# Autodesk Inventor assembly: Whales_Project
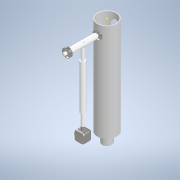
[picture p0: Inventor's stored thumbnail of the model, 180x180]
Saved by Autodesk Inventor 2020 (Build 240168000, 168)
## iProperties
Created: 2021-11-29
Part Number: Whales_Project
Document SubType Name: Assembly
Designer: Emrah BAYRAM
Author: Emrah BAYRAM
## Documents named in this file (11)
- C:\Users\umuro\OneDrive - ikc.edu.tr\Home - Library_Umur\E\Education\2020-2024_Mechatronics\Lessons\MEE203-DINAMIK\Whales_Dynamics_Project\Drawings\Assembly2.iam
- C:\Users\umuro\OneDrive - ikc.edu.tr\Home - Library_Umur\E\Education\2020-2024_Mechatronics\Lessons\MEE203-DINAMIK\Whales_Dynamics_Project\Drawings\Platform.ipt
- C:\Users\umuro\OneDrive - ikc.edu.tr\Home - Library_Umur\E\Education\2020-2024_Mechatronics\Lessons\MEE203-DINAMIK\Whales_Dynamics_Project\Drawings\Hammer.ipt
- C:\Users\umuro\OneDrive - ikc.edu.tr\Home - Library_Umur\E\Education\2020-2024_Mechatronics\Lessons\MEE203-DINAMIK\Whales_Dynamics_Project\Drawings\Marble.ipt
- C:\Users\umuro\OneDrive - ikc.edu.tr\Home - Library_Umur\E\Education\2020-2024_Mechatronics\Lessons\MEE203-DINAMIK\Whales_Dynamics_Project\Drawings\Support.ipt
- C:\Users\umuro\OneDrive - ikc.edu.tr\Home - Library_Umur\E\Education\2020-2024_Mechatronics\Lessons\MEE203-DINAMIK\Whales_Dynamics_Project\Drawings\dikey_shaft_alt.ipt
- C:\Users\umuro\OneDrive - ikc.edu.tr\Home - Library_Umur\E\Education\2020-2024_Mechatronics\Lessons\MEE203-DINAMIK\Whales_Dynamics_Project\Drawings\dikey_shaft_üst.ipt
- C:\Users\umuro\OneDrive - ikc.edu.tr\Home - Library_Umur\E\Education\2020-2024_Mechatronics\Lessons\MEE203-DINAMIK\Whales_Dynamics_Project\Drawings\shaftorj.ipt
- C:\Users\umuro\OneDrive - ikc.edu.tr\Home - Library_Umur\E\Education\2020-2024_Mechatronics\Lessons\MEE203-DINAMIK\Whales_Dynamics_Project\Drawings\shaftucu2.ipt
- C:\Users\umuro\OneDrive - ikc.edu.tr\Home - Library_Umur\E\Education\2020-2024_Mechatronics\Lessons\MEE203-DINAMIK\Whales_Dynamics_Project\Drawings\dikey_shaft.ipt
- C:\Users\umuro\OneDrive - ikc.edu.tr\Home - Library_Umur\E\Education\2020-2024_Mechatronics\Lessons\MEE203-DINAMIK\Whales_Dynamics_Project\Drawings\Assembly2\Design Accelerator\Bearing2.iam
## Components (13 placed, 10 different names)
1. Platform:1 — Mate:4, Insert:1, Mate:5, Mate:6
2. Hammer:1 — Cylindrical:4
3. Marble:1
4. Support:1 — Mate:5, Mate:6, Mate:7, Mate:9, Cylindrical:9
5. Support:2 — Mate:4, Insert:1, Mate:7, Mate:8, Cylindrical:8
6. dikey_shaft_alt:1 — Cylindrical:3, Cylindrical:4
7. dikey_shaft_üst:1 — Cylindrical:1, Cylindrical:2
8. shaftorj:1 — Cylindrical:1, Cylindrical:5, Cylindrical:6
9. shaftucu2:1 — Cylindrical:6, Mate:8
10. shaftucu2:2 — Cylindrical:5, Mate:9, Mate:10
11. dikey_shaft:1 — Cylindrical:2, Cylindrical:3
12. Bearing:1 [sub-assembly] — Mate:10, Cylindrical:9
13. Bearing:2 [sub-assembly] — Cylindrical:8
## Relationships (16: CylindricalJoint 8, Mate 7, Insert 1)
- Mate:4: Platform:1 ↔ Support:2
- Insert:1: Platform:1 ↔ Support:2
- Mate:5: Platform:1 ↔ Support:1
- Mate:6: Platform:1 ↔ Support:1
- Mate:7: Support:1 ↔ Support:2
- Cylindrical:1: dikey_shaft_üst:1 ↔ shaftorj:1
- Cylindrical:2: dikey_shaft_üst:1 ↔ dikey_shaft:1
- Cylindrical:3: dikey_shaft_alt:1 ↔ dikey_shaft:1
- Cylindrical:4: Hammer:1 ↔ dikey_shaft_alt:1
- Cylindrical:5: shaftorj:1 ↔ shaftucu2:2
- Cylindrical:6: shaftorj:1 ↔ shaftucu2:1
- Mate:8: Support:2 ↔ shaftucu2:1
- Mate:9: Support:1 ↔ shaftucu2:2
- Mate:10: shaftucu2:2 ↔ Bearing:1
- Cylindrical:8: Support:2 ↔ Bearing:2
- Cylindrical:9: Support:1 ↔ Bearing:1
## Named parameters: sa_0 = 1500, sa_1 = 0, sa_2 = 250, sa_3 = 0, sa_4 = 0, sa_5 = 250, sa_6 = 0, sa_7 = 981
note: some values were not read from the file. Shown as the stored number, unit unknown: "sa_0", "sa_1", "sa_2", "sa_3", "sa_4", "sa_5", "sa_6", "sa_7".
